# Autodesk Inventor assembly: My_Pen_Case_1pen
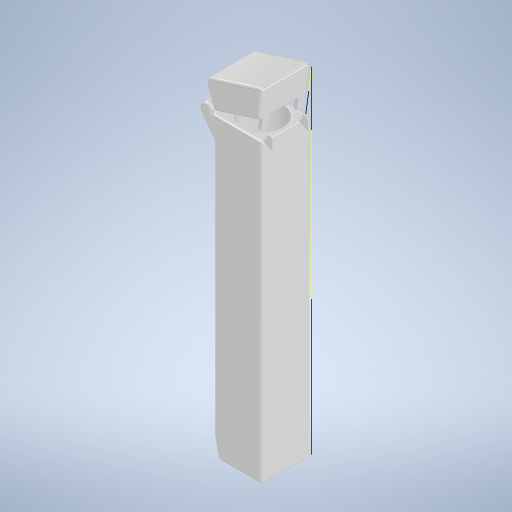
[picture p0: Inventor's stored thumbnail of the model, 512x512]
Saved by Autodesk Inventor 2024 (Build 280153000, 153)
## iProperties
Created: 2024-12-21
Part Number: My_Pen_Case_1pen
Document SubType Name: Assembly
Designer: Emil
Author: Emil
## Documents named in this file (3)
- C:\Users\Emil\OneDrive\Dokument\Projekt-Emil\Fountain_pen+Case+Pen_Holder\InventorCad\My_Pen_Cases\My_Pen_Case_1pen\My_Pen_Case_1pen.iam
- C:\Users\Emil\OneDrive\Dokument\Projekt-Emil\Fountain_pen+Case+Pen_Holder\InventorCad\My_Pen_Cases\My_Pen_Case_1pen\body_1pen.ipt
- C:\Users\Emil\OneDrive\Dokument\Projekt-Emil\Fountain_pen+Case+Pen_Holder\InventorCad\My_Pen_Cases\My_Pen_Case_1pen\Lid_1pen.ipt
## Components (2 placed, 2 different names)
1. body_1pen:1 — Insert:1
2. Lid_1pen:1 — Insert:1
## Relationships (1: Insert 1)
- Insert:1 (0.1 mm): body_1pen:1 ↔ Lid_1pen:1
